# Autodesk Inventor assembly: Tarraxa espelhada
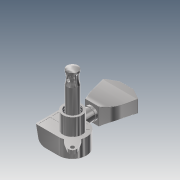
[picture p0: Inventor's stored thumbnail of the model, 180x180]
Saved by Autodesk Inventor 2016 (Build 200138000, 138)
## iProperties
Created: 2018-12-08
Part Number: Tarraxa espelhada
Document SubType Name: Assembly
Designer: Pedro Mendonça
Author: Pedro Mendonça
## Documents named in this file (4)
- C:\Users\Pedro\Google Drive\Projeto CAD Eng Mecânica\Tarraxa espelhada.iam
- C:\Users\Pedro\Google Drive\Projeto CAD Eng Mecânica\Peça 7 espelhada.ipt
- C:\Users\Pedro\Google Drive\Projeto CAD Eng Mecânica\Cabeça da tarraxa.ipt
- C:\Users\Pedro\Google Drive\Projeto CAD Eng Mecânica\Parafuso menor Tarraxa.ipt
## Components (3 placed, 3 different names)
1. Peça 7 espelhada:1 — Insert:1
2. Cabeça da tarraxa:1 — Insert:1, Insert:2
3. Parafuso menor Tarraxa:1 — Insert:2
## Relationships (2: Insert 2)
- Insert:1: Peça 7 espelhada:1 ↔ Cabeça da tarraxa:1
- Insert:2: Cabeça da tarraxa:1 ↔ Parafuso menor Tarraxa:1
